# Autodesk Inventor assembly: Bluetooth_module
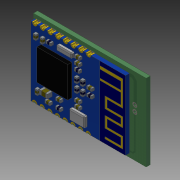
[picture p0: Inventor's stored thumbnail of the model, 180x180]
Saved by Autodesk Inventor 2013 (Build 170138000, 138)
## iProperties
Created: 2015-07-02
Part Number: Bluetooth_module
Document SubType Name: Assembly
Designer: terg
Author: terg
## Documents named in this file (6)
- C:\Users\terg\Projects\ModularElectronics\3D_models\Bluetooth_module\Bluetooth_module.iam
- C:\Users\terg\Projects\ModularElectronics\3D_models\Bluetooth_module\Bluetooth_module_PCB.ipt
- C:\Users\terg\Projects\ModularElectronics\3D_models\Bluetooth_module\HM-11.iam
- C:\Users\terg\Projects\ModularElectronics\3D_models\Components\0402_cap.ipt
- C:\Users\terg\Projects\ModularElectronics\3D_models\Components\0805_cap.ipt
- C:\Users\terg\Projects\ModularElectronics\3D_models\Components\EFM32ZG110.ipt
## Components (9 placed, 5 different names)
1. Bluetooth_module_PCB:1 — Zestawiający:1, Równoległy:1, Równoległy:2, Zestawiający:2, Zestawiający:3, Zestawiający:4, Zestawiający:5, Równoległy:3, Równoległy:4, Równoległy:5, Równoległy:6, Równoległy:7, Równoległy:8, Równoległy:9, Równoległy:10, Zestawiający:6, Zestawiający:7, Równoległy:11, Równoległy:12, Równoległy:13, Równoległy:14, Zestawiający:9, Równoległy:17, Równoległy:18
2. HM-11:1 [sub-assembly] — Zestawiający:1, Równoległy:1, Równoległy:2
3. 0402_cap:1 — Zestawiający:2, Równoległy:3, Równoległy:7
4. 0402_cap:2 — Zestawiający:3, Równoległy:6, Równoległy:10
5. 0402_cap:3 — Zestawiający:4, Równoległy:5, Równoległy:9
6. 0402_cap:4 — Zestawiający:5, Równoległy:4, Równoległy:8
7. 0805_cap:1 — Zestawiający:6, Równoległy:11, Równoległy:12
8. 0805_cap:2 — Zestawiający:7, Równoległy:13, Równoległy:14
9. EFM32ZG110:1 — Zestawiający:9, Równoległy:17, Równoległy:18
## Relationships (24: Flush 16, Mate 8)
- Zestawiający:1 [Mate]: Bluetooth_module_PCB:1 ↔ HM-11:1
- Równoległy:1 [Flush] (3.228 mm): Bluetooth_module_PCB:1 ↔ HM-11:1
- Równoległy:2 [Flush] (0.764 mm): Bluetooth_module_PCB:1 ↔ HM-11:1
- Zestawiający:2 [Mate]: Bluetooth_module_PCB:1 ↔ 0402_cap:1
- Zestawiający:3 [Mate]: Bluetooth_module_PCB:1 ↔ 0402_cap:2
- Zestawiający:4 [Mate]: Bluetooth_module_PCB:1 ↔ 0402_cap:3
- Zestawiający:5 [Mate]: Bluetooth_module_PCB:1 ↔ 0402_cap:4
- Równoległy:3 [Flush] (1.531 mm): Bluetooth_module_PCB:1 ↔ 0402_cap:1
- Równoległy:4 [Flush] (1.574 mm): Bluetooth_module_PCB:1 ↔ 0402_cap:4
- Równoległy:5 [Flush] (7.904 mm): Bluetooth_module_PCB:1 ↔ 0402_cap:3
- Równoległy:6 [Flush] (11.053 mm): Bluetooth_module_PCB:1 ↔ 0402_cap:2
- Równoległy:7 [Flush] (9.747 mm): Bluetooth_module_PCB:1 ↔ 0402_cap:1
- Równoległy:8 [Flush] (12.161 mm): Bluetooth_module_PCB:1 ↔ 0402_cap:4
- Równoległy:9 [Flush] (11.888 mm): Bluetooth_module_PCB:1 ↔ 0402_cap:3
- Równoległy:10 [Flush] (9.749 mm): Bluetooth_module_PCB:1 ↔ 0402_cap:2
- Zestawiający:6 [Mate]: Bluetooth_module_PCB:1 ↔ 0805_cap:1
- Zestawiający:7 [Mate]: Bluetooth_module_PCB:1 ↔ 0805_cap:2
- Równoległy:11 [Flush] (2.619 mm): Bluetooth_module_PCB:1 ↔ 0805_cap:1
- Równoległy:12 [Flush] (1.016 mm): Bluetooth_module_PCB:1 ↔ 0805_cap:1
- Równoległy:13 [Flush] (9.076 mm): Bluetooth_module_PCB:1 ↔ 0805_cap:2
- Równoległy:14 [Flush] (2.563 mm): Bluetooth_module_PCB:1 ↔ 0805_cap:2
- Zestawiający:9 [Mate]: Bluetooth_module_PCB:1 ↔ EFM32ZG110:1
- Równoległy:17 [Flush] (5.954 mm): Bluetooth_module_PCB:1 ↔ EFM32ZG110:1
- Równoległy:18 [Flush] (5.083 mm): Bluetooth_module_PCB:1 ↔ EFM32ZG110:1
